# Autodesk Inventor assembly: Ensamble_Soporte_Superior_Balancin
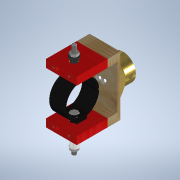
[picture p0: Inventor's stored thumbnail of the model, 180x180]
Saved by Autodesk Inventor 2022 (Build 260153000, 153)
## iProperties
Created: 2022-03-06
Part Number: Ensamble_Soporte_Superior_Balancin
Document SubType Name: Assembly
Designer: hurta
Author: hurta
## Documents named in this file (15)
- C:\Users\hurta\Documents\Universidad\NovenoSemestre\MiniProyecto1\MiniProyecto1\Diseno_Mecanico_Inventor\Ensamble_Soporte_Superior_Balancin.iam
- C:\Users\hurta\Documents\Universidad\NovenoSemestre\MiniProyecto1\MiniProyecto1\Diseno_Mecanico_Inventor\Union_Tubo_Soporte_Superior_Balancin.ipt
- C:\Users\hurta\Documents\Universidad\NovenoSemestre\MiniProyecto1\MiniProyecto1\Diseno_Mecanico_Inventor\Pieza_Ajuste_Soporte_Superior_Balancin.ipt
- C:\Users\hurta\Documents\Universidad\NovenoSemestre\MiniProyecto1\MiniProyecto1\Diseno_Mecanico_Inventor\Ajuste_Soporte_Cojinete.ipt
- C:\Users\hurta\Documents\Universidad\NovenoSemestre\MiniProyecto1\MiniProyecto1\Diseno_Mecanico_Inventor\Soporte_Superior_Cojinete.ipt
- C:\Users\hurta\Documents\Universidad\NovenoSemestre\MiniProyecto1\MiniProyecto1\Diseno_Mecanico_Inventor\Cojinete.ipt
- C:\Users\hurta\Documents\Universidad\NovenoSemestre\MiniProyecto1\MiniProyecto1\Diseno_Mecanico_Inventor\Soporte_PVC_Union_Balancin.ipt
- C:\Users\hurta\Documents\Universidad\NovenoSemestre\MiniProyecto1\MiniProyecto1\Diseno_Mecanico_Inventor\Adaptador_Perno_Cojinete.ipt
- C:\Users\hurta\Documents\Universidad\NovenoSemestre\MiniProyecto1\MiniProyecto1\Diseno_Mecanico_Inventor\libreria\en-US\AS 1111\AS 1111 - M8 x 50.ipt
- C:\Users\hurta\Documents\Universidad\NovenoSemestre\MiniProyecto1\MiniProyecto1\Diseno_Mecanico_Inventor\libreria\en-US\AS 1111\AS 1111 - M8 x 65.ipt
- C:\Users\hurta\Documents\Universidad\NovenoSemestre\MiniProyecto1\MiniProyecto1\Diseno_Mecanico_Inventor\Transmision_Potencia\polea8m.ipt
- C:\Users\hurta\Documents\Universidad\NovenoSemestre\MiniProyecto1\MiniProyecto1\Diseno_Mecanico_Inventor\libreria\en-US\AS 1112 (4)\AS 1112 - M8(2).ipt
- C:\Users\hurta\Documents\Universidad\NovenoSemestre\MiniProyecto1\MiniProyecto1\Diseno_Mecanico_Inventor\libreria\en-US\AS 1110\AS 1110 - M5 x 16.ipt
- C:\Users\hurta\Documents\Universidad\NovenoSemestre\MiniProyecto1\MiniProyecto1\Diseno_Mecanico_Inventor\libreria\en-US\AS 1112 (4)\AS 1112 - M5(2).ipt
- C:\Users\hurta\Documents\Universidad\NovenoSemestre\MiniProyecto1\MiniProyecto1\Diseno_Mecanico_Inventor\libreria\en-US\AS 1110\AS 1110 - M4 x 30.ipt
## Components (28 placed, 14 different names)
1. Union_Tubo_Soporte_Superior_Balancin:1 — Mate:1, Mate:2, Mate:3, Mate:61, Mate:62
2. Pieza_Ajuste_Soporte_Superior_Balancin:1 — Mate:1, Mate:2, Mate:3, Mate:10, Mate:11, Mate:12, Mate:19, Mate:20, Mate:21, Mate:47, Mate:48, Mate:49, Mate:50, Mate:51, Mate:52, Mate:53, Mate:54, Mate:55, Mate:56, Mate:57, Mate:58
3. Ajuste_Soporte_Cojinete:1 — Mate:14, Mate:16, Mate:18, Mate:20, Mate:21, Mate:22, Mate:23, Mate:24
4. Ajuste_Soporte_Cojinete:2 — Mate:13, Mate:14, Mate:15, Mate:16, Mate:17, Mate:18
5. Ajuste_Soporte_Cojinete:3 — Mate:13, Mate:15, Mate:17, Mate:19
6. Ajuste_Soporte_Cojinete:4 — Mate:4, Mate:7, Mate:9, Mate:10, Mate:11, Mate:25, Mate:26
7. Ajuste_Soporte_Cojinete:5 — Mate:4, Mate:5, Mate:6, Mate:8, Mate:12
8. Ajuste_Soporte_Cojinete:6 — Mate:5, Mate:6, Mate:7, Mate:8, Mate:9
9. Soporte_Superior_Cojinete:1 — Flush:1, Mate:22, Mate:23, Mate:24, Mate:30
10. Soporte_Superior_Cojinete:2 — Flush:1, Mate:25, Mate:26, Mate:28, Mate:29
11. Cojinete:1 — Mate:27, Mate:30, Mate:31, Mate:32, Mate:33, Mate:34
12. Cojinete:2 — Mate:27, Mate:28, Mate:29, Mate:35, Mate:36
13. Soporte_PVC_Union_Balancin:1 — Mate:31, Mate:32, Mate:38, Mate:40
14. Adaptador_Perno_Cojinete:1 — Mate:33, Mate:34, Mate:37, Mate:46
15. Adaptador_Perno_Cojinete:2 — Mate:35, Mate:36, Mate:39, Mate:42
16. AS 1111 - Metric M8 x 50:1 — Mate:37, Mate:38, Mate:45
17. AS 1111 - Metric M8 x 65:1 — Mate:39, Mate:40, Mate:41, Mate:43
18. polea8m:1 — Mate:41, Mate:42, Mate:44
19. AS 1112 (4) - Metric M8:1 — Mate:43, Mate:44
20. AS 1112 (4) - Metric M8:2 — Mate:45, Mate:46
21. AS 1110 - Metric M4 x 30:1 — Mate:47, Mate:53
22. AS 1110 - Metric M4 x 30:2 — Mate:49, Mate:52
23. AS 1110 - Metric M4 x 30:3 — Mate:48, Mate:54
24. AS 1110 - Metric M4 x 30:4 — Mate:50, Mate:51
25. AS 1110 - Metric M5 x 16:1 — Mate:55, Mate:58, Mate:59
26. AS 1110 - Metric M5 x 16:2 — Mate:56, Mate:57, Mate:60
27. AS 1112 (4) - Metric M5:1 — Mate:59, Mate:61
28. AS 1112 (4) - Metric M5:2 — Mate:60, Mate:62
## Relationships (63: Mate 62, Flush 1)
- Mate:1: Union_Tubo_Soporte_Superior_Balancin:1 ↔ Pieza_Ajuste_Soporte_Superior_Balancin:1
- Mate:2: Union_Tubo_Soporte_Superior_Balancin:1 ↔ Pieza_Ajuste_Soporte_Superior_Balancin:1
- Mate:3: Union_Tubo_Soporte_Superior_Balancin:1 ↔ Pieza_Ajuste_Soporte_Superior_Balancin:1
- Mate:4: Ajuste_Soporte_Cojinete:4 ↔ Ajuste_Soporte_Cojinete:5
- Mate:5: Ajuste_Soporte_Cojinete:5 ↔ Ajuste_Soporte_Cojinete:6
- Mate:6: Ajuste_Soporte_Cojinete:5 ↔ Ajuste_Soporte_Cojinete:6
- Mate:7: Ajuste_Soporte_Cojinete:4 ↔ Ajuste_Soporte_Cojinete:6
- Mate:8: Ajuste_Soporte_Cojinete:5 ↔ Ajuste_Soporte_Cojinete:6
- Mate:9: Ajuste_Soporte_Cojinete:4 ↔ Ajuste_Soporte_Cojinete:6
- Mate:10: Pieza_Ajuste_Soporte_Superior_Balancin:1 ↔ Ajuste_Soporte_Cojinete:4
- Mate:11: Pieza_Ajuste_Soporte_Superior_Balancin:1 ↔ Ajuste_Soporte_Cojinete:4
- Mate:12: Pieza_Ajuste_Soporte_Superior_Balancin:1 ↔ Ajuste_Soporte_Cojinete:5
- Mate:13: Ajuste_Soporte_Cojinete:2 ↔ Ajuste_Soporte_Cojinete:3
- Mate:14: Ajuste_Soporte_Cojinete:1 ↔ Ajuste_Soporte_Cojinete:2
- Mate:15: Ajuste_Soporte_Cojinete:2 ↔ Ajuste_Soporte_Cojinete:3
- Mate:16: Ajuste_Soporte_Cojinete:1 ↔ Ajuste_Soporte_Cojinete:2
- Mate:17: Ajuste_Soporte_Cojinete:2 ↔ Ajuste_Soporte_Cojinete:3
- Mate:18: Ajuste_Soporte_Cojinete:1 ↔ Ajuste_Soporte_Cojinete:2
- Mate:19: Pieza_Ajuste_Soporte_Superior_Balancin:1 ↔ Ajuste_Soporte_Cojinete:3
- Mate:20: Pieza_Ajuste_Soporte_Superior_Balancin:1 ↔ Ajuste_Soporte_Cojinete:1
- Mate:21: Pieza_Ajuste_Soporte_Superior_Balancin:1 ↔ Ajuste_Soporte_Cojinete:1
- Flush:1: Soporte_Superior_Cojinete:1 ↔ Soporte_Superior_Cojinete:2
- Mate:22: Ajuste_Soporte_Cojinete:1 ↔ Soporte_Superior_Cojinete:1
- Mate:23: Ajuste_Soporte_Cojinete:1 ↔ Soporte_Superior_Cojinete:1
- Mate:24: Ajuste_Soporte_Cojinete:1 ↔ Soporte_Superior_Cojinete:1
- Mate:25: Ajuste_Soporte_Cojinete:4 ↔ Soporte_Superior_Cojinete:2
- Mate:26: Ajuste_Soporte_Cojinete:4 ↔ Soporte_Superior_Cojinete:2
- Mate:27: Cojinete:1 ↔ Cojinete:2
- Mate:28: Soporte_Superior_Cojinete:2 ↔ Cojinete:2
- Mate:29: Soporte_Superior_Cojinete:2 ↔ Cojinete:2
- Mate:30: Soporte_Superior_Cojinete:1 ↔ Cojinete:1
- Mate:31: Cojinete:1 ↔ Soporte_PVC_Union_Balancin:1
- Mate:32 (1.4 mm): Cojinete:1 ↔ Soporte_PVC_Union_Balancin:1
- Mate:33: Cojinete:1 ↔ Adaptador_Perno_Cojinete:1
- Mate:34: Cojinete:1 ↔ Adaptador_Perno_Cojinete:1
- Mate:35: Cojinete:2 ↔ Adaptador_Perno_Cojinete:2
- Mate:36: Cojinete:2 ↔ Adaptador_Perno_Cojinete:2
- Mate:37: Adaptador_Perno_Cojinete:1 ↔ AS 1111 - Metric M8 x 50:1
- Mate:38: Soporte_PVC_Union_Balancin:1 ↔ AS 1111 - Metric M8 x 50:1
- Mate:39: Adaptador_Perno_Cojinete:2 ↔ AS 1111 - Metric M8 x 65:1
- Mate:40: Soporte_PVC_Union_Balancin:1 ↔ AS 1111 - Metric M8 x 65:1
- Mate:41: AS 1111 - Metric M8 x 65:1 ↔ polea8m:1
- Mate:42: Adaptador_Perno_Cojinete:2 ↔ polea8m:1
- Mate:43: AS 1111 - Metric M8 x 65:1 ↔ AS 1112 (4) - Metric M8:1
- Mate:44: polea8m:1 ↔ AS 1112 (4) - Metric M8:1
- Mate:45: AS 1111 - Metric M8 x 50:1 ↔ AS 1112 (4) - Metric M8:2
- Mate:46: Adaptador_Perno_Cojinete:1 ↔ AS 1112 (4) - Metric M8:2
- Mate:47: Pieza_Ajuste_Soporte_Superior_Balancin:1 ↔ AS 1110 - Metric M4 x 30:1
- Mate:48: Pieza_Ajuste_Soporte_Superior_Balancin:1 ↔ AS 1110 - Metric M4 x 30:3
- Mate:49: Pieza_Ajuste_Soporte_Superior_Balancin:1 ↔ AS 1110 - Metric M4 x 30:2
- Mate:50: Pieza_Ajuste_Soporte_Superior_Balancin:1 ↔ AS 1110 - Metric M4 x 30:4
- Mate:51: Pieza_Ajuste_Soporte_Superior_Balancin:1 ↔ AS 1110 - Metric M4 x 30:4
- Mate:52: Pieza_Ajuste_Soporte_Superior_Balancin:1 ↔ AS 1110 - Metric M4 x 30:2
- Mate:53: Pieza_Ajuste_Soporte_Superior_Balancin:1 ↔ AS 1110 - Metric M4 x 30:1
- Mate:54: Pieza_Ajuste_Soporte_Superior_Balancin:1 ↔ AS 1110 - Metric M4 x 30:3
- Mate:55: Pieza_Ajuste_Soporte_Superior_Balancin:1 ↔ AS 1110 - Metric M5 x 16:1
- Mate:56: Pieza_Ajuste_Soporte_Superior_Balancin:1 ↔ AS 1110 - Metric M5 x 16:2
- Mate:57: Pieza_Ajuste_Soporte_Superior_Balancin:1 ↔ AS 1110 - Metric M5 x 16:2
- Mate:58: Pieza_Ajuste_Soporte_Superior_Balancin:1 ↔ AS 1110 - Metric M5 x 16:1
- Mate:59: AS 1110 - Metric M5 x 16:1 ↔ AS 1112 (4) - Metric M5:1
- Mate:60: AS 1110 - Metric M5 x 16:2 ↔ AS 1112 (4) - Metric M5:2
- Mate:61: Union_Tubo_Soporte_Superior_Balancin:1 ↔ AS 1112 (4) - Metric M5:1
- Mate:62: Union_Tubo_Soporte_Superior_Balancin:1 ↔ AS 1112 (4) - Metric M5:2
